# Autodesk Inventor assembly: Assy_arm_connection
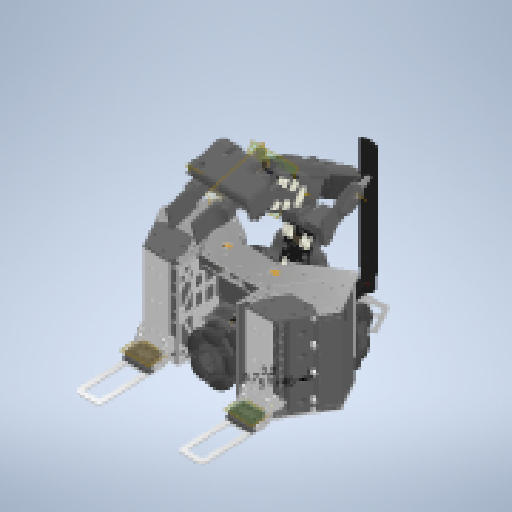
[picture p0: Inventor's stored thumbnail of the model, 512x512]
Saved by Autodesk Inventor 2024.1 (Build 281209000, 209)
## iProperties
Created: 2025-03-04
Part Number: Assy_arm_connection
Document SubType Name: Assembly
Designer: hibik
Author: hibik
## Documents named in this file (3)
- C:\Users\hibik\Documents\Robomech\RESCUE\ORCA\hard\Assy_arm_connection.iam
- C:\Users\hibik\Documents\Robomech\RESCUE\ORCA\hard\Assy_fork_connection.iam
- C:\Users\hibik\Documents\Robomech\RESCUE\ORCA\hard\arm\Assy_arm.iam
## Components (2 placed, 2 different names)
1. Assy_fork_connection:1 [sub-assembly] — 正接:1, 角度:1, メイト:1
2. Assy_arm:1 [sub-assembly] — 正接:1, 角度:1, メイト:1
## Relationships (3: Tangent 1, Angle 1, Mate 1)
- 正接:1 [Tangent]: Assy_fork_connection:1 ↔ Assy_arm:1
- 角度:1 [Angle] (180 deg): Assy_fork_connection:1 ↔ Assy_arm:1
- メイト:1 [Mate] (1 mm): Assy_fork_connection:1 ↔ Assy_arm:1
